# Autodesk Inventor assembly: bottomarm
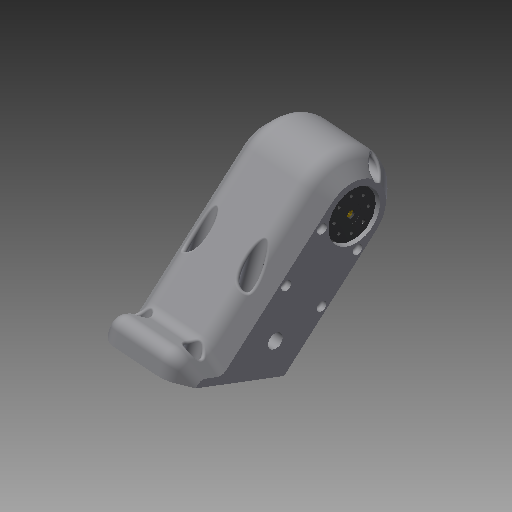
[picture p0: Inventor's stored thumbnail of the model, 512x512]
Saved by Autodesk Inventor 2018 (Build 220112000, 112)
## iProperties
Created: 2018-02-04
Part Number: bottomarm
Document SubType Name: Assembly
Designer: Clevo
Author: Clevo
## Documents named in this file (3)
- E:\RobotArm\bottomarm.iam
- E:\RobotArm\LX-16A.iam
- E:\RobotArm\arm1.ipt
## Components (2 placed, 2 different names)
1. LX-16A:1 [sub-assembly] — Mate:3
2. arm1:1 — Mate:3
## Relationships (3: Mate 2, Angle 1)
- [Mate]: LX-16A:1 ↔ arm1:1
- [Angle] (0 deg): LX-16A:1 ↔ arm1:1
- Mate:3: LX-16A:1 ↔ arm1:1
